# Autodesk Inventor assembly: clip and shaft assem
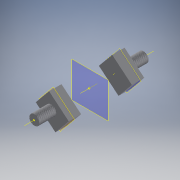
[picture p0: Inventor's stored thumbnail of the model, 180x180]
Saved by Autodesk Inventor 2019.3 (Build 233278000, 278)
## iProperties
Created: 2018-12-21
Part Number: clip and shaft assem
Document SubType Name: Assembly
Designer: Frienddo
Author: Frienddo
## Documents named in this file (4)
- D:\hive\projects\pocketpelvis\models\mounts\V2\femur\clip and shaft assem.iam
- D:\hive\projects\pocketpelvis\models\mounts\V2\femur\shaft toothed clip toothed v2.ipt
- D:\hive\projects\pocketpelvis\models\mounts\V2\femur\shaft toothed.ipt
- D:\hive\projects\pocketpelvis\models\mounts\V2\femur\shaft toothed clip holder v2 hole bool.ipt
## Components (6 placed, 3 different names)
1. shaft toothed clip toothed v2:1 — Mate:4, Mate:5, Flush:1, Flush:3, Symmetry:1, Flush:7, Flush:8, Flush:9
2. shaft toothed:1 — Mate:2, Flush:3
3. shaft toothed:2 — Mate:1, Mate:2, Flush:2
4. shaft toothed clip toothed v2:2 — Mate:3, Mate:4, Mate:5, Flush:1, Flush:2, Symmetry:1, Flush:4, Flush:5, Flush:6
5. shaft toothed clip holder v2 hole bool:1 — Flush:4, Flush:5, Flush:6
6. shaft toothed clip holder v2 hole bool:2 — Flush:7, Flush:8, Flush:9
## Relationships (17: Flush 9, Mate 7, Symmetry 1)
- Mate:1: shaft toothed:2
- Mate:2: shaft toothed:1 ↔ shaft toothed:2
- Mate:3: shaft toothed clip toothed v2:2
- Mate:4: shaft toothed clip toothed v2:1 ↔ shaft toothed clip toothed v2:2
- Mate:5 (-77.963 mm): shaft toothed clip toothed v2:1 ↔ shaft toothed clip toothed v2:2
- Flush:1: shaft toothed clip toothed v2:1 ↔ shaft toothed clip toothed v2:2
- Flush:2: shaft toothed:2 ↔ shaft toothed clip toothed v2:2
- Flush:3: shaft toothed clip toothed v2:1 ↔ shaft toothed:1
- Symmetry:1: shaft toothed clip toothed v2:1 ↔ shaft toothed clip toothed v2:2
- Mate:6
- Mate:7
- Flush:4 (-0.25 mm): shaft toothed clip toothed v2:2 ↔ shaft toothed clip holder v2 hole bool:1
- Flush:5 (-0.25 mm): shaft toothed clip toothed v2:2 ↔ shaft toothed clip holder v2 hole bool:1
- Flush:6 (-0.25 mm): shaft toothed clip toothed v2:2 ↔ shaft toothed clip holder v2 hole bool:1
- Flush:7 (-0.25 mm): shaft toothed clip toothed v2:1 ↔ shaft toothed clip holder v2 hole bool:2
- Flush:8 (-0.25 mm): shaft toothed clip toothed v2:1 ↔ shaft toothed clip holder v2 hole bool:2
- Flush:9 (-0.25 mm): shaft toothed clip toothed v2:1 ↔ shaft toothed clip holder v2 hole bool:2
## Named parameters: ballDist = 77.963 mm
